# Autodesk Inventor assembly: Lupfer von oben assembly
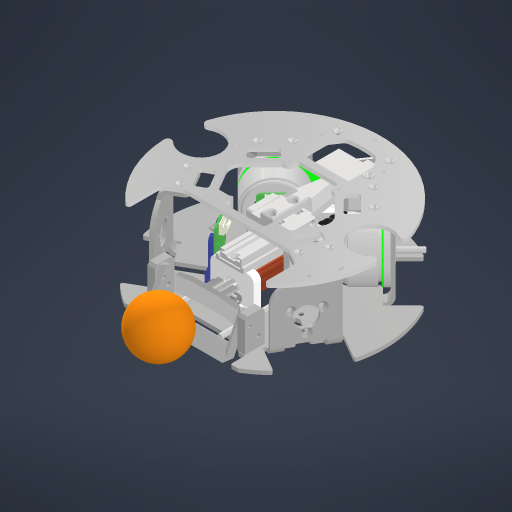
[picture p0: Inventor's stored thumbnail of the model, 512x512]
Saved by Autodesk Inventor 2024.2 (Build 282272000, 272)
## iProperties
Created: 2023-12-02
Part Number: Lupfer von oben assembly
Document SubType Name: Assembly
Designer: jacob
Author: jacob
## Documents named in this file (32)
- C:\Users\Lukas\Nextcloud\2.3 - Mechanik - Soccer\Entwicklungs Sandboxes\Lukas Waldhoff\Bot_Gen1\Lupfer\Lupfer_assambly_Jacob_2.0\Lupfer assembly.iam
- C:\Users\Lukas\Nextcloud\2.3 - Mechanik - Soccer\Entwicklungs Sandboxes\Lukas Waldhoff\Bot_Gen1\Lupfer\Lupfer_assambly_Jacob_2.0\igus_schine.ipt
- C:\Users\Lukas\Nextcloud\2.3 - Mechanik - Soccer\Entwicklungs Sandboxes\Lukas Waldhoff\Bot_Gen1\Lupfer\Lupfer_assambly_Jacob_2.0\Igus Gleiter.ipt
- C:\Users\Lukas\Nextcloud\2.3 - Mechanik - Soccer\Entwicklungs Sandboxes\Lukas Waldhoff\Bot_Gen1\Lupfer\Lupfer_assambly_Jacob_2.0\Lupfer oben.ipt
- C:\Users\Lukas\Nextcloud\2.3 - Mechanik - Soccer\Entwicklungs Sandboxes\Lukas Waldhoff\Bot_Gen1\Lupfer\Lupfer_assambly_Jacob_2.0\Stoßstange.ipt
- C:\Users\Lukas\Nextcloud\2.3 - Mechanik - Soccer\Entwicklungs Sandboxes\Lukas Waldhoff\Bot_Gen1\Lupfer\Lupfer_assambly_Jacob_2.0\Laeufer.iam
- C:\Users\Lukas\Nextcloud\2.3 - Mechanik - Soccer\Entwicklungs Sandboxes\Lukas Waldhoff\Bot_Gen1\Lupfer\Lupfer_assambly_Jacob_2.0\Zwischenplatte.ipt
- C:\Users\Lukas\Nextcloud\2.3 - Mechanik - Soccer\Entwicklungs Sandboxes\Lukas Waldhoff\Bot_Gen1\Lupfer\Lupfer_assambly_Jacob_2.0\Hülse zum einhaken.ipt
- C:\Users\Lukas\Nextcloud\2.3 - Mechanik - Soccer\Entwicklungs Sandboxes\Lukas Waldhoff\Bot_Gen1\Lupfer\Lupfer_assambly_Jacob_2.0\Golfball.ipt
- C:\Users\Lukas\Nextcloud\2.3 - Mechanik - Soccer\Entwicklungs Sandboxes\Lukas Waldhoff\Bot_Gen1\Lupfer\Lupfer_assambly_Jacob_2.0\Halterrung_Stange.ipt
- C:\Users\Lukas\Nextcloud\2.3 - Mechanik - Soccer\Entwicklungs Sandboxes\Lukas Waldhoff\Bot_Gen1\Lupfer\Lupfer_assambly_Jacob_2.0\Stange halter.ipt
- C:\Users\Lukas\Nextcloud\2.3 - Mechanik - Soccer\Entwicklungs Sandboxes\Lukas Waldhoff\Bot_Gen1\Lupfer\Lupfer_assambly_Jacob_2.0\Grundplatte_Bordeaux_modifiziert.ipt
- C:\Users\Lukas\Nextcloud\2.3 - Mechanik - Soccer\Entwicklungs Sandboxes\Lukas Waldhoff\Bot_Gen1\Lupfer\Lupfer_assambly_Jacob_2.0\DF45L024048-A.iam
- C:\Users\Lukas\Nextcloud\2.3 - Mechanik - Soccer\Entwicklungs Sandboxes\Lukas Waldhoff\Bot_Gen1\Lupfer\Lupfer_assambly_Jacob_2.0\Lupfer Seite.ipt
- C:\Users\Lukas\Nextcloud\2.3 - Mechanik - Soccer\Entwicklungs Sandboxes\Lukas Waldhoff\Bot_Gen1\Lupfer\Lupfer_assambly_Jacob_2.0\First_Floor_aktuell v35.ipt
- C:\Users\Lukas\Nextcloud\2.3 - Mechanik - Soccer\Entwicklungs Sandboxes\Lukas Waldhoff\Bot_Gen1\Lupfer\Lupfer_assambly_Jacob_2.0\Motor.ipt
- C:\Users\Lukas\Nextcloud\2.3 - Mechanik - Soccer\Entwicklungs Sandboxes\Lukas Waldhoff\Bot_Gen1\Lupfer\Lupfer_assambly_Jacob_2.0\Motor Adapter.ipt
- C:\Users\Lukas\Nextcloud\2.3 - Mechanik - Soccer\Entwicklungs Sandboxes\Lukas Waldhoff\Bot_Gen1\Lupfer\Lupfer_assambly_Jacob_2.0\motor halterrung.ipt
- C:\Users\Lukas\Nextcloud\2.3 - Mechanik - Soccer\Entwicklungs Sandboxes\Lukas Waldhoff\Bot_Gen1\Lupfer\Lupfer_assambly_Jacob_2.0\Magnet.ipt
- C:\Users\Lukas\Nextcloud\2.3 - Mechanik - Soccer\Entwicklungs Sandboxes\Lukas Waldhoff\Bot_Gen1\Lupfer\Lupfer_assambly_Jacob_2.0\Magnet-arm.ipt
- C:\Users\Lukas\Nextcloud\2.3 - Mechanik - Soccer\Entwicklungs Sandboxes\Lukas Waldhoff\Bot_Gen1\Lupfer\Lupfer_assambly_Jacob_2.0\Stoßstange_MIR.ipt
- C:\Users\Lukas\Nextcloud\2.3 - Mechanik - Soccer\Entwicklungs Sandboxes\Lukas Waldhoff\Bot_Gen1\Lupfer\Lupfer_assambly_Jacob_2.0\Lupferschaufel innen v2\Lupferschaufel innen v2.ipt
- C:\Users\Lukas\Nextcloud\2.3 - Mechanik - Soccer\Entwicklungs Sandboxes\Lukas Waldhoff\Bot_Gen1\Lupfer\Lupfer_assambly_Jacob_2.0\Dribblerhalterung v10.ipt
- C:\Users\Lukas\Nextcloud\2.3 - Mechanik - Soccer\Entwicklungs Sandboxes\Lukas Waldhoff\Bot_Gen1\Lupfer\Lupfer_assambly_Jacob_2.0\Lupfer Seite_MIR1.ipt
- C:\Users\Lukas\Nextcloud2\2.3 - Mechanik - Soccer\Entwicklungs Sandboxes\Lukas Waldhoff\Bot_Gen1\Lupfer\Lupfer_assambly_Jacob_2.0\Encoderhalter3_Lupfer_Kompatibel v3\Encoderhalter3_Lupfer_Kompatibel.iam
- C:\Users\Lukas\Nextcloud2\2.3 - Mechanik - Soccer\Entwicklungs Sandboxes\Lukas Waldhoff\Bot_Gen1\Lupfer\Lupfer_assambly_Jacob_2.0\652203A2.ipt
- C:\Users\Lukas\Nextcloud2\2.3 - Mechanik - Soccer\Entwicklungs Sandboxes\Lukas Waldhoff\Bot_Gen1\Lupfer\Lupfer_assambly_Jacob_2.0\Endkappe plus Federhalter 3D.ipt
- C:\Users\Lukas\Nextcloud2\2.3 - Mechanik - Soccer\Entwicklungs Sandboxes\Lukas Waldhoff\Bot_Gen1\Lupfer\Lupfer_assambly_Jacob_2.0\Endcap_Lupfercompatibel_vorne.ipt
- C:\Users\Lukas\Nextcloud\2.3 - Mechanik - Soccer\Entwicklungs Sandboxes\Lukas Waldhoff\Bot_Gen1\Lupfer\Lupfer_assambly_Jacob_2.0\Hüllse mit Isolator.ipt
- C:\Users\Lukas\Nextcloud\2.3 - Mechanik - Soccer\Entwicklungs Sandboxes\Lukas Waldhoff\Bot_Gen1\Lupfer\Lupfer_assambly_Jacob_2.0\Capinsert_back.ipt
- C:\Users\Lukas\Nextcloud\2.3 - Mechanik - Soccer\Entwicklungs Sandboxes\Lukas Waldhoff\Bot_Gen1\Lupfer\Lupfer_assambly_Jacob_2.0\Spule.ipt
- C:\Users\Lukas\Nextcloud\2.3 - Mechanik - Soccer\Entwicklungs Sandboxes\Lukas Waldhoff\Bot_Gen1\Lupfer\Lupfer_assambly_Jacob_2.0\Capinsert_front.ipt
## Components (38 placed, 31 different names)
1. igus_schine:1 — Passend:1, Passend:2, Einfügen:60, Einfügen:61
2. Igus Gleiter:1 — Passend:1, Passend:2, Einfügen:48, Einfügen:49
3. Lupfer oben:1 — Passend:19, Einfügen:43, Einfügen:48, Einfügen:49, Einfügen:62, Winkel:6, Einfügen:64, Winkel:8
4. Stoßstange:2 — Einfügen:42
5. Laeufer:1 [sub-assembly] — Einfügen:7, Passend:55, Passend:56, Winkel:7
6. Zwischenplatte:1 — Passend:52, Einfügen:59, Passend:53, Einfügen:60, Einfügen:61
7. Hülse zum einhaken:1 — Einfügen:7, Passend:54
8. Golfball:1 — Passend:40
9. Halterrung_Stange:1 — Passend:19, Einfügen:16, Passend:54, Tangential:1
10. Stange halter:1 — Einfügen:62, Tangential:1
11. Grundplatte_Bordeaux_modifiziert:1 — Einfügen:10, Einfügen:11, Winkel:3, Winkel:4, Einfügen:13, Einfügen:14, Passend:26, Passend:27, Passend:28, Fluchtend:35, Fluchtend:36, Passend:34, Einfügen:36, Einfügen:37, Einfügen:38, Einfügen:39, Passend:40, Einfügen:51, Einfügen:52, Einfügen:53, Einfügen:54, Passend:44, Passend:45, Passend:46, Passend:48, Passend:49, Passend:51, Winkel:7
12. DF45L024048-A:1 [sub-assembly] — Einfügen:10, Winkel:4
13. DF45L024048-A:2 [sub-assembly] — Einfügen:11, Winkel:3
14. Lupfer Seite:1 — Einfügen:42, Einfügen:43, Winkel:6
15. First_Floor_aktuell v35:1 — Einfügen:13, Einfügen:14, Winkel:5, Passend:32
16. Motor:1 — Passend:26, Passend:27, Winkel:5, Einfügen:15, Passend:28, Passend:30, Passend:31
17. Motor Adapter:1 — Einfügen:15, Einfügen:34, Einfügen:35
18. motor halterrung:1 — Passend:30, Passend:31, Passend:32
19. Magnet:1 — Einfügen:16
20. Magnet:2 — Einfügen:17
21. Magnet-arm:1 — Einfügen:17, Einfügen:34, Einfügen:35
22. Stoßstange_MIR:1 — Einfügen:45
23. Lupferschaufel innen v2:1 — Einfügen:40
24. Dribblerhalterung v10:1 — Einfügen:38, Einfügen:39
25. Dribblerhalterung v10:2 — Einfügen:36, Einfügen:37, Einfügen:40
26. Lupfer Seite_MIR1:1 — Einfügen:45, Einfügen:64, Winkel:8
27. Encoderhalter3_Lupfer_Kompatibel:1 [sub-assembly] — Einfügen:51, Einfügen:52
28. Encoderhalter3_Lupfer_Kompatibel:2 [sub-assembly] — Einfügen:53, Einfügen:54, Einfügen:55, Einfügen:56, Einfügen:57, Einfügen:58
29. 652203A2:1 — Einfügen:55
30. 652203A2:2 — Einfügen:58
31. 652203A2:3 — Einfügen:57
32. 652203A2:4 — Einfügen:56
33. Endkappe plus Federhalter 3D:1 — Passend:44, Passend:45, Passend:46, Einfügen:59, Passend:53
34. Endcap_Lupfercompatibel_vorne:1 — Passend:48, Passend:49, Passend:51, Passend:52, Passend:63, Passend:64, Passend:65
35. Hüllse mit Isolator:1 — Einfügen:63, Passend:57, Passend:58, Passend:59, Passend:60, Passend:61, Passend:62
36. Capinsert_back:1 — Passend:60, Passend:61, Passend:62
37. Spule:1 — Passend:55, Passend:56, Einfügen:63
38. Capinsert_front:1 — Passend:57, Passend:58, Passend:59, Passend:63, Passend:64, Passend:65
## Relationships (74: Insert 34, Mate 31, Angle 6, Flush 2, Tangent 1)
- Passend:1 [Mate]: igus_schine:1 ↔ Igus Gleiter:1
- Passend:2 [Mate]: igus_schine:1 ↔ Igus Gleiter:1
- Einfügen:7 [Insert]: Laeufer:1 ↔ Hülse zum einhaken:1
- Passend:19 [Mate]: Lupfer oben:1 ↔ Halterrung_Stange:1
- Einfügen:10 [Insert]: Grundplatte_Bordeaux_modifiziert:1 ↔ DF45L024048-A:1
- Einfügen:11 [Insert]: Grundplatte_Bordeaux_modifiziert:1 ↔ DF45L024048-A:2
- Winkel:3 [Angle] (-90 deg): Grundplatte_Bordeaux_modifiziert:1 ↔ DF45L024048-A:2
- Winkel:4 [Angle] (-90 deg): Grundplatte_Bordeaux_modifiziert:1 ↔ DF45L024048-A:1
- Einfügen:13 [Insert]: Grundplatte_Bordeaux_modifiziert:1 ↔ First_Floor_aktuell v35:1
- Einfügen:14 [Insert]: Grundplatte_Bordeaux_modifiziert:1 ↔ First_Floor_aktuell v35:1
- Passend:26 [Mate] (1 mm): Grundplatte_Bordeaux_modifiziert:1 ↔ Motor:1
- Passend:27 [Mate]: Grundplatte_Bordeaux_modifiziert:1 ↔ Motor:1
- Winkel:5 [Angle] (0 deg): First_Floor_aktuell v35:1 ↔ Motor:1
- Einfügen:15 [Insert]: Motor:1 ↔ Motor Adapter:1
- Passend:28 [Mate] (2 mm): Grundplatte_Bordeaux_modifiziert:1 ↔ Motor:1
- Passend:30 [Mate]: Motor:1 ↔ motor halterrung:1
- Passend:31 [Mate]: Motor:1 ↔ motor halterrung:1
- Passend:32 [Mate]: First_Floor_aktuell v35:1 ↔ motor halterrung:1
- Einfügen:16 [Insert]: Halterrung_Stange:1 ↔ Magnet:1
- Einfügen:17 [Insert]: Magnet:2 ↔ Magnet-arm:1
- Fluchtend:35 [Flush]: Grundplatte_Bordeaux_modifiziert:1
- Fluchtend:36 [Flush]: Grundplatte_Bordeaux_modifiziert:1
- Passend:34 [Mate]: Grundplatte_Bordeaux_modifiziert:1
- Einfügen:34 [Insert]: Motor Adapter:1 ↔ Magnet-arm:1
- Einfügen:35 [Insert]: Motor Adapter:1 ↔ Magnet-arm:1
- Einfügen:36 [Insert]: Grundplatte_Bordeaux_modifiziert:1 ↔ Dribblerhalterung v10:2
- Einfügen:37 [Insert]: Grundplatte_Bordeaux_modifiziert:1 ↔ Dribblerhalterung v10:2
- Einfügen:38 [Insert]: Grundplatte_Bordeaux_modifiziert:1 ↔ Dribblerhalterung v10:1
- Einfügen:39 [Insert]: Grundplatte_Bordeaux_modifiziert:1 ↔ Dribblerhalterung v10:1
- Einfügen:40 [Insert] (0.75 mm): Lupferschaufel innen v2:1 ↔ Dribblerhalterung v10:2
- Passend:40 [Mate] (-16.5 mm): Golfball:1 ↔ Grundplatte_Bordeaux_modifiziert:1
- Einfügen:42 [Insert]: Stoßstange:2 ↔ Lupfer Seite:1
- Einfügen:43 [Insert]: Lupfer oben:1 ↔ Lupfer Seite:1
- Einfügen:45 [Insert]: Stoßstange_MIR:1 ↔ Lupfer Seite_MIR1:1
- Einfügen:48 [Insert]: Igus Gleiter:1 ↔ Lupfer oben:1
- Einfügen:49 [Insert]: Igus Gleiter:1 ↔ Lupfer oben:1
- Einfügen:51 [Insert]: Grundplatte_Bordeaux_modifiziert:1 ↔ Encoderhalter3_Lupfer_Kompatibel:1
- Einfügen:52 [Insert]: Grundplatte_Bordeaux_modifiziert:1 ↔ Encoderhalter3_Lupfer_Kompatibel:1
- Einfügen:53 [Insert]: Grundplatte_Bordeaux_modifiziert:1 ↔ Encoderhalter3_Lupfer_Kompatibel:2
- Einfügen:54 [Insert]: Grundplatte_Bordeaux_modifiziert:1 ↔ Encoderhalter3_Lupfer_Kompatibel:2
- Einfügen:55 [Insert]: Encoderhalter3_Lupfer_Kompatibel:2 ↔ 652203A2:1
- Einfügen:56 [Insert]: Encoderhalter3_Lupfer_Kompatibel:2 ↔ 652203A2:4
- Einfügen:57 [Insert]: Encoderhalter3_Lupfer_Kompatibel:2 ↔ 652203A2:3
- Einfügen:58 [Insert]: Encoderhalter3_Lupfer_Kompatibel:2 ↔ 652203A2:2
- Passend:44 [Mate]: Grundplatte_Bordeaux_modifiziert:1 ↔ Endkappe plus Federhalter 3D:1
- Passend:45 [Mate]: Grundplatte_Bordeaux_modifiziert:1 ↔ Endkappe plus Federhalter 3D:1
- Passend:46 [Mate] (0.1 mm): Grundplatte_Bordeaux_modifiziert:1 ↔ Endkappe plus Federhalter 3D:1
- Passend:48 [Mate]: Grundplatte_Bordeaux_modifiziert:1 ↔ Endcap_Lupfercompatibel_vorne:1
- Passend:49 [Mate] (0.1 mm): Grundplatte_Bordeaux_modifiziert:1 ↔ Endcap_Lupfercompatibel_vorne:1
- Passend:51 [Mate]: Grundplatte_Bordeaux_modifiziert:1 ↔ Endcap_Lupfercompatibel_vorne:1
- Passend:52 [Mate]: Zwischenplatte:1 ↔ Endcap_Lupfercompatibel_vorne:1
- Einfügen:59 [Insert]: Zwischenplatte:1 ↔ Endkappe plus Federhalter 3D:1
- Passend:53 [Mate]: Zwischenplatte:1 ↔ Endkappe plus Federhalter 3D:1
- Einfügen:60 [Insert]: igus_schine:1 ↔ Zwischenplatte:1
- Einfügen:61 [Insert]: igus_schine:1 ↔ Zwischenplatte:1
- Passend:54 [Mate]: Hülse zum einhaken:1 ↔ Halterrung_Stange:1
- Einfügen:62 [Insert]: Lupfer oben:1 ↔ Stange halter:1
- Tangential:1: Halterrung_Stange:1 ↔ Stange halter:1
- Winkel:6 [Angle] (1 deg): Lupfer oben:1 ↔ Lupfer Seite:1
- Passend:55 [Mate]: Laeufer:1 ↔ Spule:1
- Passend:56 [Mate]: Laeufer:1 ↔ Spule:1
- Winkel:7 [Angle] (180 deg): Laeufer:1 ↔ Grundplatte_Bordeaux_modifiziert:1
- Einfügen:63 [Insert]: Hüllse mit Isolator:1 ↔ Spule:1
- Passend:57 [Mate]: Hüllse mit Isolator:1 ↔ Capinsert_front:1
- Passend:58 [Mate]: Hüllse mit Isolator:1 ↔ Capinsert_front:1
- Passend:59 [Mate]: Hüllse mit Isolator:1 ↔ Capinsert_front:1
- Passend:60 [Mate]: Hüllse mit Isolator:1 ↔ Capinsert_back:1
- Passend:61 [Mate]: Hüllse mit Isolator:1 ↔ Capinsert_back:1
- Passend:62 [Mate]: Hüllse mit Isolator:1 ↔ Capinsert_back:1
- Passend:63 [Mate]: Endcap_Lupfercompatibel_vorne:1 ↔ Capinsert_front:1
- Passend:64 [Mate]: Endcap_Lupfercompatibel_vorne:1 ↔ Capinsert_front:1
- Passend:65 [Mate]: Endcap_Lupfercompatibel_vorne:1 ↔ Capinsert_front:1
- Einfügen:64 [Insert]: Lupfer oben:1 ↔ Lupfer Seite_MIR1:1
- Winkel:8 [Angle] (-1 deg): Lupfer oben:1 ↔ Lupfer Seite_MIR1:1
